# Autodesk Inventor assembly: CIM motor 12T for 446
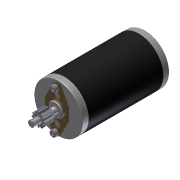
[picture p0: Inventor's stored thumbnail of the model, 180x180]
Saved by Autodesk Inventor 2013 (Build 170138000, 138)
## iProperties
Created: 2012-10-14
Part Number: CIM motor 12T for 446
Document SubType Name: Assembly
Designer: Nemo
Author: Nemo
## Documents named in this file (4)
- H:\Nemo\Documents\Robotics\COTS Parts\Motors\CIM motor 12T for 446.iam
- H:\Nemo\Documents\Robotics\COTS Parts\Motors\CIM motor 12T for AM Shifters.iam
- H:\Nemo\Documents\Robotics\COTS Parts\Gearboxes\Spacers\CIM Spacer 125.ipt
- H:\Nemo\Documents\Robotics\COTS Parts\Fasteners\10-32 SHCS x750.ipt
## Components (4 placed, 3 different names)
1. CIM motor 12T for AM Shifters:1 [sub-assembly]
2. CIM Spacer 125:1
3. 10-32 SHCS x750:1
4. 10-32 SHCS x750:2
## Relationships (4: Insert 3, Mate 1)
- [Insert]: CIM motor 12T for AM Shifters:1 ↔ CIM Spacer 125:1
- [Mate]: CIM motor 12T for AM Shifters:1 ↔ CIM Spacer 125:1
- [Insert] (3.175 mm): CIM Spacer 125:1 ↔ 10-32 SHCS x750:2
- [Insert] (3.175 mm): CIM Spacer 125:1 ↔ 10-32 SHCS x750:1
